# Autodesk Inventor assembly: Złożenie
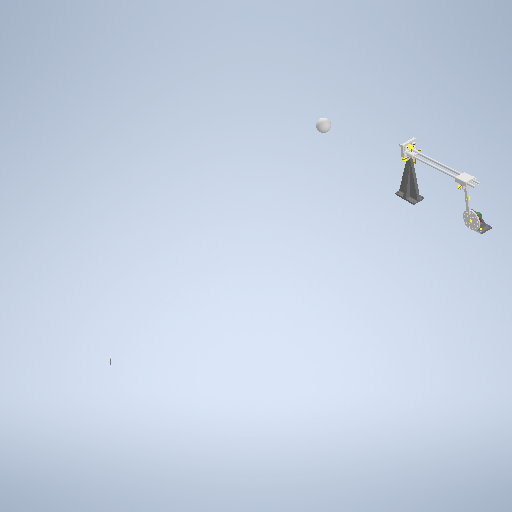
[picture p0: Inventor's stored thumbnail of the model, 512x512]
Saved by Autodesk Inventor 2025.2 (Build 292293000, 293)
## iProperties
Created: 2025-11-25
Part Number: Złożenie
Document SubType Name: Assembly
Designer: juras
Author: juras
## Documents named in this file (15)
- C:\Users\juras\Desktop\AiR SEMESTRY\AiR SEMESTR 5\SYSTEMY MIKROPROCESOROWE\LABORATORIUM\PROJEKT_KULKA_PID\KULKA_PID_KONSTRUKCJA\Złożenie.iam
- C:\Users\juras\Desktop\AiR SEMESTRY\AiR SEMESTR 5\SYSTEMY MIKROPROCESOROWE\LABORATORIUM\PROJEKT_KULKA_PID\KULKA_PID_KONSTRUKCJA\DO_DRUKU_3D\Servo_podstawa.ipt
- C:\Users\juras\Desktop\AiR SEMESTRY\AiR SEMESTR 5\SYSTEMY MIKROPROCESOROWE\LABORATORIUM\PROJEKT_KULKA_PID\KULKA_PID_KONSTRUKCJA\SG90_SG90\SG90_SG90\SG90_SG90.iam
- C:\Users\juras\Desktop\AiR SEMESTRY\AiR SEMESTR 5\SYSTEMY MIKROPROCESOROWE\LABORATORIUM\PROJEKT_KULKA_PID\KULKA_PID_KONSTRUKCJA\SG90_Arm_04_Custom\SG90_Arm_04_Custom\SG90_Arm_04_Custom.ipt
- C:\Users\juras\Desktop\AiR SEMESTRY\AiR SEMESTR 5\SYSTEMY MIKROPROCESOROWE\LABORATORIUM\PROJEKT_KULKA_PID\KULKA_PID_KONSTRUKCJA\DO_DRUKU_3D\Servo_przelozenie.ipt
- C:\Users\juras\Desktop\AiR SEMESTRY\AiR SEMESTR 5\SYSTEMY MIKROPROCESOROWE\LABORATORIUM\PROJEKT_KULKA_PID\KULKA_PID_KONSTRUKCJA\DO_DRUKU_3D\Czujnik_podstawa.ipt
- C:\Users\juras\Desktop\AiR SEMESTRY\AiR SEMESTR 5\SYSTEMY MIKROPROCESOROWE\LABORATORIUM\PROJEKT_KULKA_PID\KULKA_PID_KONSTRUKCJA\DO_DRUKU_3D\Toweript.ipt
- C:\Users\juras\Desktop\AiR SEMESTRY\AiR SEMESTR 5\SYSTEMY MIKROPROCESOROWE\LABORATORIUM\PROJEKT_KULKA_PID\KULKA_PID_KONSTRUKCJA\piłka.ipt
- C:\Users\juras\Desktop\AiR SEMESTRY\AiR SEMESTR 5\SYSTEMY MIKROPROCESOROWE\LABORATORIUM\PROJEKT_KULKA_PID\KULKA_PID_KONSTRUKCJA\DO_DRUKU_3D\szpilka.ipt
- C:\Users\juras\Desktop\AiR SEMESTRY\AiR SEMESTR 5\SYSTEMY MIKROPROCESOROWE\LABORATORIUM\PROJEKT_KULKA_PID\KULKA_PID_KONSTRUKCJA\DO_DRUKU_3D\zaslepka.ipt
- C:\Users\juras\Desktop\AiR SEMESTRY\AiR SEMESTR 5\SYSTEMY MIKROPROCESOROWE\LABORATORIUM\PROJEKT_KULKA_PID\KULKA_PID_KONSTRUKCJA\HC-SR04 Sensor\HC-SR04 Sensor\HC-SR04 Sensor.ipt
- C:\Users\juras\Desktop\AiR SEMESTRY\AiR SEMESTR 5\SYSTEMY MIKROPROCESOROWE\LABORATORIUM\PROJEKT_KULKA_PID\KULKA_PID_KONSTRUKCJA\DO_DRUKU_3D\element_posredni.ipt
- C:\Users\juras\Desktop\AiR SEMESTRY\AiR SEMESTR 5\SYSTEMY MIKROPROCESOROWE\LABORATORIUM\PROJEKT_KULKA_PID\KULKA_PID_KONSTRUKCJA\DO_DRUKU_3D\sworzen.ipt
- C:\Users\juras\Desktop\AiR SEMESTRY\AiR SEMESTR 5\SYSTEMY MIKROPROCESOROWE\LABORATORIUM\PROJEKT_KULKA_PID\KULKA_PID_KONSTRUKCJA\DO_DRUKU_3D\sruba_m2.ipt
- C:\Users\juras\Desktop\AiR SEMESTRY\AiR SEMESTR 5\SYSTEMY MIKROPROCESOROWE\LABORATORIUM\PROJEKT_KULKA_PID\KULKA_PID_KONSTRUKCJA\DO_DRUKU_3D\nakretka_m2.ipt
## Components (17 placed, 14 different names)
1. Servo_podstawa:1 — Zestawiające:1, Zestawiające:2, Równoległe:1, Zestawiające:3, Zestawiające:4, Zestawiające:5, Równoległe:2
2. SG90_SG90:1 [sub-assembly] — Zestawiające:3, Zestawiające:4, Zestawiające:5, Zestawiające:6, Zestawiające:7
3. SG90_Arm_04_Custom:1 — Zestawiające:6, Zestawiające:7, Zestawiające:45, Zestawiające:46
4. Toweript:1 — Równoległe:2, Zestawiające:54, Zestawiające:55
5. piłka:1
6. zaslepka:1 — Zestawiające:47, Zestawiające:48, Zestawiające:60, Zestawiające:61, Zestawiające:62, Zestawiające:63
7. Servo_przelozenie:2 — Zestawiające:45, Zestawiające:46, Zestawiające:49, Zestawiające:50
8. element_posredni:1 — Zestawiające:47, Zestawiające:48, Zestawiające:49, Zestawiające:50
9. Czujnik_podstawa:1 — Zestawiające:51, Zestawiające:52, Zestawiające:53, Zestawiające:54, Zestawiające:55, Zestawiające:56, Zestawiające:57, Zestawiające:58, Zestawiające:59, Zestawiające:64, Zestawiające:65, Zestawiające:66, Zestawiające:67, Zestawiające:69
10. HC-SR04 Sensor:1 — Zestawiające:51, Zestawiające:52, Zestawiające:53
11. szpilka:1 — Zestawiające:56, Zestawiające:57, Zestawiające:61
12. szpilka:2 — Zestawiające:58, Zestawiające:59, Zestawiające:60
13. sworzen:1 — Zestawiające:62, Zestawiające:63
14. sworzen:2 — Zestawiające:64, Zestawiające:65
15. sruba_m2:1
16. sruba_m2:2 — Zestawiające:66, Zestawiające:67, Zestawiające:68
17. nakretka_m2:1 — Zestawiające:68, Zestawiające:69
## Relationships (34: Mate 32, Flush 2)
- Zestawiające:1 [Mate] (-27.5 mm): Servo_podstawa:1
- Zestawiające:2 [Mate] (-30 mm): Servo_podstawa:1
- Równoległe:1 [Flush] (20 mm): Servo_podstawa:1
- Zestawiające:3 [Mate]: Servo_podstawa:1 ↔ SG90_SG90:1
- Zestawiające:4 [Mate] (1 mm): Servo_podstawa:1 ↔ SG90_SG90:1
- Zestawiające:5 [Mate]: Servo_podstawa:1 ↔ SG90_SG90:1
- Zestawiające:6 [Mate]: SG90_SG90:1 ↔ SG90_Arm_04_Custom:1
- Zestawiające:7 [Mate] (1 mm): SG90_SG90:1 ↔ SG90_Arm_04_Custom:1
- Równoległe:2 [Flush]: Servo_podstawa:1 ↔ Toweript:1
- Zestawiające:45 [Mate]: SG90_Arm_04_Custom:1 ↔ Servo_przelozenie:2
- Zestawiające:46 [Mate]: SG90_Arm_04_Custom:1 ↔ Servo_przelozenie:2
- Zestawiające:47 [Mate]: zaslepka:1 ↔ element_posredni:1
- Zestawiające:48 [Mate]: zaslepka:1 ↔ element_posredni:1
- Zestawiające:49 [Mate]: Servo_przelozenie:2 ↔ element_posredni:1
- Zestawiające:50 [Mate]: Servo_przelozenie:2 ↔ element_posredni:1
- Zestawiające:51 [Mate]: Czujnik_podstawa:1 ↔ HC-SR04 Sensor:1
- Zestawiające:52 [Mate]: Czujnik_podstawa:1 ↔ HC-SR04 Sensor:1
- Zestawiające:53 [Mate]: Czujnik_podstawa:1 ↔ HC-SR04 Sensor:1
- Zestawiające:54 [Mate]: Toweript:1 ↔ Czujnik_podstawa:1
- Zestawiające:55 [Mate]: Toweript:1 ↔ Czujnik_podstawa:1
- Zestawiające:56 [Mate]: Czujnik_podstawa:1 ↔ szpilka:1
- Zestawiające:57 [Mate]: Czujnik_podstawa:1 ↔ szpilka:1
- Zestawiające:58 [Mate]: Czujnik_podstawa:1 ↔ szpilka:2
- Zestawiające:59 [Mate]: Czujnik_podstawa:1 ↔ szpilka:2
- Zestawiające:60 [Mate]: zaslepka:1 ↔ szpilka:2
- Zestawiające:61 [Mate]: zaslepka:1 ↔ szpilka:1
- Zestawiające:62 [Mate]: zaslepka:1 ↔ sworzen:1
- Zestawiające:63 [Mate] (2 mm): zaslepka:1 ↔ sworzen:1
- Zestawiające:64 [Mate]: Czujnik_podstawa:1 ↔ sworzen:2
- Zestawiające:65 [Mate]: Czujnik_podstawa:1 ↔ sworzen:2
- Zestawiające:66 [Mate]: Czujnik_podstawa:1 ↔ sruba_m2:2
- Zestawiające:67 [Mate]: Czujnik_podstawa:1 ↔ sruba_m2:2
- Zestawiające:68 [Mate]: sruba_m2:2 ↔ nakretka_m2:1
- Zestawiające:69 [Mate] (2 mm): Czujnik_podstawa:1 ↔ nakretka_m2:1
